# Autodesk Inventor assembly: 0002_Part_De_xe
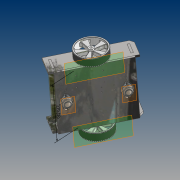
[picture p0: Inventor's stored thumbnail of the model, 180x180]
Saved by Autodesk Inventor 2021 (Build 250183000, 183)
## iProperties
Created: 2024-04-07
Part Number: 0002_Part_De_xe
Document SubType Name: Assembly
Designer: Admin
Mass: 20745.8 g
Surface Area: 9003.08 cm^2
Volume: 3062.25 cm^3
Density: 6.77468 g/cm^3
Author: Admin
## Documents named in this file (17)
- C:\Users\Admin\Desktop\DO_AN_TOT_NGHIEP_2024\Mechanical\Design_in_3D\Version_2\0002_Part_De_xe.iam
- C:\Users\Admin\Desktop\DO_AN_TOT_NGHIEP_2024\Mechanical\Design_in_3D\Version_1\0001_ASS_Hop_so.iam
- C:\Users\Admin\Desktop\DO_AN_TOT_NGHIEP_2024\Mechanical\Design_in_3D\Version_2\01_Tam_de_01.ipt
- C:\Users\Admin\Desktop\DO_AN_TOT_NGHIEP_2024\Mechanical\Design_in_3D\Version_2\02_Tam_hong.ipt
- C:\Users\Admin\Desktop\DO_AN_TOT_NGHIEP_2024\Mechanical\Design_in_3D\Version_2\03_Tam_top_vs_bottom.ipt
- C:\Users\Admin\Desktop\Do_an\Ver_3\Thu_vien\67060-roller-ball-bearing-1.snapshot.1\67060, ROLLER BALL BEARING.iam
- C:\Users\Admin\Desktop\DO_AN_TOT_NGHIEP_2024\Mechanical\Design_in_3D\Version_2\04_Mieng_go_dem_lo_xo.ipt
- C:\Users\Admin\Desktop\DO_AN_TOT_NGHIEP_2024\Mechanical\Design_in_3D\Library\lineare-bearing-lmuu-complete-serie-1.snapshot.3\Lineare_bearing_LMUU_serie_LM6UU.ipt
- C:\Users\Admin\Desktop\DO_AN_TOT_NGHIEP_2024\Mechanical\Design_in_3D\Version_2\05_Tam_truot_lo_xo.ipt
- C:\Users\Admin\Documents\Inventor\Content Center Files\R2021\en-US\BS EN ISO 7045 Z\EN ISO 7045 - M6 x 60 - 4.8 - Z(1).ipt
- C:\Users\Admin\Desktop\DO_AN_TOT_NGHIEP_2024\Mechanical\Design_in_3D\Library\Lo_xo_phi_7x40.ipt
- C:\Users\Admin\Desktop\DO_AN_TOT_NGHIEP_2024\Mechanical\Design_in_3D\Version_2\06_Truc_phi_6x70.ipt
- C:\Users\Admin\Desktop\DO_AN_TOT_NGHIEP_2024\Mechanical\Design_in_3D\Version_2\07_Co_dinh_cay_nen_lo_xo.ipt
- C:\Users\Admin\Documents\Inventor\Content Center Files\R2021\en-US\AS 1971 (M - 5)\AS 1971 - 6(1).ipt
- C:\Users\Admin\Desktop\DO_AN_TOT_NGHIEP_2024\Mechanical\Design_in_3D\Version_2\12_Tam_go_top.ipt
- C:\Users\Admin\Desktop\DO_AN_TOT_NGHIEP_2024\Mechanical\Design_in_3D\Version_2\03_Tam_mat_truoc.ipt
- C:\Users\Admin\Desktop\Do_an\Ver_4\001_Ban_le.ipt
## Components (38 placed, 16 different names)
1. 0001_ASS_Hop_so:1 [sub-assembly] — Mate:1, Flush:1, Mate:2, Symmetry:1, Mate:12, Mate:40, Mate:53
2. 0001_ASS_Hop_so:2 [sub-assembly] — Mate:1, Flush:1, Mate:2, Mate:4, Symmetry:1, Mate:52
3. 01_Tam_de_01:1 — Mate:4, Mate:5, Mate:7, Flush:4, Flush:5, Mate:11, Insert:1, Mate:15, Insert:5, Mate:32, Mate:40, Mate:55, Mate:56, Mate:59, Mate:62, Mate:64, Mate:67, Mate:69, Mate:72, Mate:75, Mate:81
4. 03_Tam_top_vs_bottom:1 — Flush:7, Mate:11, Mate:49, Mate:50, Flush:12, Mate:58, Mate:66, Mate:70, Mate:79
5. 02_Tam_hong:2 — Mate:7, Flush:4, Flush:5, Flush:7, Flush:13, Mate:63, Mate:65, Mate:68, Mate:77, Mate:78, Mate:79
6. 67060, ROLLER BALL BEARING:1 [sub-assembly] — Mate:12, Mate:16, Mate:17, Flush:8, Flush:10, Mate:52
7. 04_Mieng_go_dem_lo_xo:1 — Insert:1, Mate:15, Mate:16, Mate:17, Mate:18, Mate:19, Insert:4, Mate:29, Mate:31
8. Lineare_bearing_LMUU_serie_LM6UU:1 — Mate:20, Mate:25
9. 05_Tam_truot_lo_xo:1 — Mate:18, Mate:19, Mate:20, Insert:2, Insert:3, Mate:25
10. BS EN ISO 7045 Z - Metric M6 x 60 - 4.8 - Z:1 — Insert:2, Mate:21, Flush:8, Mate:28
11. BS EN ISO 7045 Z - Metric M6 x 60 - 4.8 - Z:2 — Insert:3, Mate:23, Mate:30
12. Lo_xo_phi_7x40:1 — Mate:21, Mate:42
13. Lo_xo_phi_7x40:2 — Mate:23, Mate:41
14. 06_Truc_phi_6x70:1 — Insert:4, Mate:26, Flush:9
15. 07_Co_dinh_cay_nen_lo_xo:1 — Mate:26, Flush:9, Flush:11
16. AS 1971 (M - 5) 6:1 — Mate:28, Mate:29, Mate:41, Mate:42
17. AS 1971 (M - 5) 6:2 — Mate:30, Mate:31
18. 04_Mieng_go_dem_lo_xo:2 — Insert:5, Mate:32, Insert:8, Mate:44
19. Lineare_bearing_LMUU_serie_LM6UU:2 — Mate:39
20. 05_Tam_truot_lo_xo:2 — Mate:43, Mate:45
21. BS EN ISO 7045 Z - Metric M6 x 60 - 4.8 - Z:3 — Mate:47
22. BS EN ISO 7045 Z - Metric M6 x 60 - 4.8 - Z:4 — Mate:44, Mate:46
23. Lo_xo_phi_7x40:3 — Mate:43
24. Lo_xo_phi_7x40:4 — Mate:45
25. 06_Truc_phi_6x70:2 — Mate:39, Insert:8, Mate:48
26. 67060, ROLLER BALL BEARING:2 [sub-assembly] — Mate:46, Mate:47, Flush:10, Mate:53
27. 07_Co_dinh_cay_nen_lo_xo:2 — Mate:48, Mate:49, Flush:11
28. 12_Tam_go_top:1 — Mate:50, Flush:12
29. 03_Tam_mat_truoc:1 — Flush:13, Mate:55, Mate:61, Mate:73, Mate:76, Mate:78, Mate:80, Mate:82
30. 001_Ban_le:1 — Mate:56, Mate:58, Flush:14
31. 001_Ban_le:2 — Mate:62, Mate:63, Flush:14
32. 001_Ban_le:3 — Mate:64, Mate:65, Flush:15
33. 001_Ban_le:4 — Mate:59, Mate:61, Flush:15
34. 001_Ban_le:5 — Mate:72, Mate:73
35. 001_Ban_le:6 — Mate:66, Mate:67, Mate:68
36. 001_Ban_le:7 — Mate:69, Mate:70
37. 001_Ban_le:8 — Mate:75, Mate:76, Mate:77
38. 02_Tam_hong:3 — Mate:80, Mate:81, Mate:82
## Relationships (85: Mate 64, Flush 12, Insert 8, Symmetry 1)
- Mate:1: 0001_ASS_Hop_so:1 ↔ 0001_ASS_Hop_so:2
- Flush:1: 0001_ASS_Hop_so:1 ↔ 0001_ASS_Hop_so:2
- Mate:2 (10 mm): 0001_ASS_Hop_so:1 ↔ 0001_ASS_Hop_so:2
- Mate:4: 0001_ASS_Hop_so:2 ↔ 01_Tam_de_01:1
- Symmetry:1: 0001_ASS_Hop_so:1 ↔ 0001_ASS_Hop_so:2
- Mate:5: 01_Tam_de_01:1
- Mate:7: 01_Tam_de_01:1 ↔ 02_Tam_hong:2
- Flush:4: 01_Tam_de_01:1 ↔ 02_Tam_hong:2
- Flush:5: 01_Tam_de_01:1 ↔ 02_Tam_hong:2
- Flush:7: 03_Tam_top_vs_bottom:1 ↔ 02_Tam_hong:2
- Mate:11: 01_Tam_de_01:1 ↔ 03_Tam_top_vs_bottom:1
- Mate:12: 0001_ASS_Hop_so:1 ↔ 67060, ROLLER BALL BEARING:1
- Insert:1: 01_Tam_de_01:1 ↔ 04_Mieng_go_dem_lo_xo:1
- Mate:15: 01_Tam_de_01:1 ↔ 04_Mieng_go_dem_lo_xo:1
- Mate:16: 67060, ROLLER BALL BEARING:1 ↔ 04_Mieng_go_dem_lo_xo:1
- Mate:17: 67060, ROLLER BALL BEARING:1 ↔ 04_Mieng_go_dem_lo_xo:1
- Mate:18: 04_Mieng_go_dem_lo_xo:1 ↔ 05_Tam_truot_lo_xo:1
- Mate:19: 04_Mieng_go_dem_lo_xo:1 ↔ 05_Tam_truot_lo_xo:1
- Mate:20: Lineare_bearing_LMUU_serie_LM6UU:1 ↔ 05_Tam_truot_lo_xo:1
- Insert:2: 05_Tam_truot_lo_xo:1 ↔ BS EN ISO 7045 Z - Metric M6 x 60 - 4.8 - Z:1
- Insert:3: 05_Tam_truot_lo_xo:1 ↔ BS EN ISO 7045 Z - Metric M6 x 60 - 4.8 - Z:2
- Mate:21: BS EN ISO 7045 Z - Metric M6 x 60 - 4.8 - Z:1 ↔ Lo_xo_phi_7x40:1
- Mate:23: BS EN ISO 7045 Z - Metric M6 x 60 - 4.8 - Z:2 ↔ Lo_xo_phi_7x40:2
- Flush:8 (-10 mm): 67060, ROLLER BALL BEARING:1 ↔ BS EN ISO 7045 Z - Metric M6 x 60 - 4.8 - Z:1
- Insert:4: 04_Mieng_go_dem_lo_xo:1 ↔ 06_Truc_phi_6x70:1
- Mate:25: Lineare_bearing_LMUU_serie_LM6UU:1 ↔ 05_Tam_truot_lo_xo:1
- Mate:26: 06_Truc_phi_6x70:1 ↔ 07_Co_dinh_cay_nen_lo_xo:1
- Flush:9 (5 mm): 06_Truc_phi_6x70:1 ↔ 07_Co_dinh_cay_nen_lo_xo:1
- Mate:28: BS EN ISO 7045 Z - Metric M6 x 60 - 4.8 - Z:1 ↔ AS 1971 (M - 5) 6:1
- Mate:29: 04_Mieng_go_dem_lo_xo:1 ↔ AS 1971 (M - 5) 6:1
- Mate:30: BS EN ISO 7045 Z - Metric M6 x 60 - 4.8 - Z:2 ↔ AS 1971 (M - 5) 6:2
- Mate:31: 04_Mieng_go_dem_lo_xo:1 ↔ AS 1971 (M - 5) 6:2
- Insert:5: 01_Tam_de_01:1 ↔ 04_Mieng_go_dem_lo_xo:2
- Mate:32: 01_Tam_de_01:1 ↔ 04_Mieng_go_dem_lo_xo:2
- [Mate]: Lineare_bearing_LMUU_serie_LM6UU:2 ↔ 05_Tam_truot_lo_xo:2
- [Insert]: 05_Tam_truot_lo_xo:2 ↔ BS EN ISO 7045 Z - Metric M6 x 60 - 4.8 - Z:3
- [Insert]: 05_Tam_truot_lo_xo:2 ↔ BS EN ISO 7045 Z - Metric M6 x 60 - 4.8 - Z:4
- [Mate]: BS EN ISO 7045 Z - Metric M6 x 60 - 4.8 - Z:3 ↔ Lo_xo_phi_7x40:3
- [Mate]: BS EN ISO 7045 Z - Metric M6 x 60 - 4.8 - Z:4 ↔ Lo_xo_phi_7x40:4
- [Mate]: Lineare_bearing_LMUU_serie_LM6UU:2 ↔ 05_Tam_truot_lo_xo:2
- Mate:39: Lineare_bearing_LMUU_serie_LM6UU:2 ↔ 06_Truc_phi_6x70:2
- Mate:40: 0001_ASS_Hop_so:1 ↔ 01_Tam_de_01:1
- Mate:41: Lo_xo_phi_7x40:2 ↔ AS 1971 (M - 5) 6:1
- Mate:42: Lo_xo_phi_7x40:1 ↔ AS 1971 (M - 5) 6:1
- Insert:8: 04_Mieng_go_dem_lo_xo:2 ↔ 06_Truc_phi_6x70:2
- Mate:43: 05_Tam_truot_lo_xo:2 ↔ Lo_xo_phi_7x40:3
- Mate:44: 04_Mieng_go_dem_lo_xo:2 ↔ BS EN ISO 7045 Z - Metric M6 x 60 - 4.8 - Z:4
- Mate:45: 05_Tam_truot_lo_xo:2 ↔ Lo_xo_phi_7x40:4
- Mate:46: BS EN ISO 7045 Z - Metric M6 x 60 - 4.8 - Z:4 ↔ 67060, ROLLER BALL BEARING:2
- Mate:47: BS EN ISO 7045 Z - Metric M6 x 60 - 4.8 - Z:3 ↔ 67060, ROLLER BALL BEARING:2
- Flush:10: 67060, ROLLER BALL BEARING:1 ↔ 67060, ROLLER BALL BEARING:2
- Mate:48: 06_Truc_phi_6x70:2 ↔ 07_Co_dinh_cay_nen_lo_xo:2
- Mate:49: 03_Tam_top_vs_bottom:1 ↔ 07_Co_dinh_cay_nen_lo_xo:2
- Flush:11: 07_Co_dinh_cay_nen_lo_xo:1 ↔ 07_Co_dinh_cay_nen_lo_xo:2
- Mate:50: 03_Tam_top_vs_bottom:1 ↔ 12_Tam_go_top:1
- Flush:12: 03_Tam_top_vs_bottom:1 ↔ 12_Tam_go_top:1
- Mate:52: 0001_ASS_Hop_so:2 ↔ 67060, ROLLER BALL BEARING:1
- Mate:53: 0001_ASS_Hop_so:1 ↔ 67060, ROLLER BALL BEARING:2
- Flush:13: 02_Tam_hong:2 ↔ 03_Tam_mat_truoc:1
- Mate:55: 01_Tam_de_01:1 ↔ 03_Tam_mat_truoc:1
- Mate:56: 01_Tam_de_01:1 ↔ 001_Ban_le:1
- Mate:58 (20 mm): 03_Tam_top_vs_bottom:1 ↔ 001_Ban_le:1
- Mate:59: 01_Tam_de_01:1 ↔ 001_Ban_le:4
- Mate:61 (20 mm): 03_Tam_mat_truoc:1 ↔ 001_Ban_le:4
- Mate:62: 01_Tam_de_01:1 ↔ 001_Ban_le:2
- Mate:63: 02_Tam_hong:2 ↔ 001_Ban_le:2
- Flush:14: 001_Ban_le:1 ↔ 001_Ban_le:2
- Mate:64: 01_Tam_de_01:1 ↔ 001_Ban_le:3
- Mate:65: 02_Tam_hong:2 ↔ 001_Ban_le:3
- Flush:15: 001_Ban_le:3 ↔ 001_Ban_le:4
- Mate:66: 03_Tam_top_vs_bottom:1 ↔ 001_Ban_le:6
- Mate:67: 01_Tam_de_01:1 ↔ 001_Ban_le:6
- Mate:68 (30 mm): 02_Tam_hong:2 ↔ 001_Ban_le:6
- Mate:69: 01_Tam_de_01:1 ↔ 001_Ban_le:7
- Mate:70: 03_Tam_top_vs_bottom:1 ↔ 001_Ban_le:7
- Mate:72: 01_Tam_de_01:1 ↔ 001_Ban_le:5
- Mate:73: 03_Tam_mat_truoc:1 ↔ 001_Ban_le:5
- Mate:75: 01_Tam_de_01:1 ↔ 001_Ban_le:8
- Mate:76: 03_Tam_mat_truoc:1 ↔ 001_Ban_le:8
- Mate:77 (30 mm): 02_Tam_hong:2 ↔ 001_Ban_le:8
- Mate:78: 02_Tam_hong:2 ↔ 03_Tam_mat_truoc:1
- Mate:79: 03_Tam_top_vs_bottom:1 ↔ 02_Tam_hong:2
- Mate:80: 03_Tam_mat_truoc:1 ↔ 02_Tam_hong:3
- Mate:81: 01_Tam_de_01:1 ↔ 02_Tam_hong:3
- Mate:82: 03_Tam_mat_truoc:1 ↔ 02_Tam_hong:3
## Named parameters: d53_d43 = 0 mm, d54_d33 = 0 mm, d55_d34 = 0 mm, d56_d35 = 0 mm, d57_d36 = 0 mm, d59_d38 = 0 mm
